# Autodesk Inventor assembly: AxisX
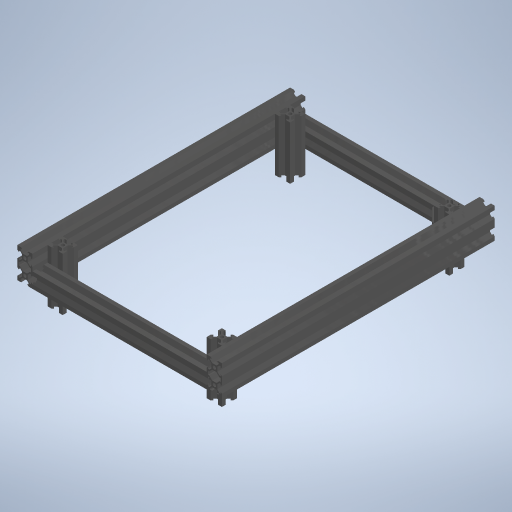
[picture p0: Inventor's stored thumbnail of the model, 512x512]
Saved by Autodesk Inventor 2024.2 (Build 282272000, 272)
## iProperties
Created: 2024-08-26
Part Number: AxisX
Document SubType Name: Assembly
Designer: Admin
Author: Admin
## Documents named in this file (5)
- C:\Users\Admin\Documents\GitHub\ManipuladorCartesiano\DiseñoMecánico\Assemblies\AxisX.iam
- C:\Users\Admin\Documents\GitHub\ManipuladorCartesiano\DiseñoMecánico\Axis\AxisX\AP-X1.ipt
- C:\Users\Admin\Documents\GitHub\ManipuladorCartesiano\DiseñoMecánico\Axis\AxisX\AP-X2.ipt
- C:\Users\Admin\Documents\GitHub\ManipuladorCartesiano\DiseñoMecánico\Axis\AxisX\AP-Support.ipt
- C:\Users\Admin\Documents\GitHub\ManipuladorCartesiano\DiseñoMecánico\AuxiliarPieces\Bracket 2020\CornerBracket2020.ipt
## Components (10 placed, 4 different names)
1. AP-X1:1 — Mate:1, Flush:1, Flush:2, Mate:3, Flush:5, Flush:8, Mate:7, Flush:10, Mate:12
2. AP-X1:2 — Mate:2, Flush:3, Flush:4, Mate:4, Flush:6, Mate:6, Flush:7, Flush:9, Mate:10, Mate:15
3. AP-X2:1 — Mate:3, Mate:4, Flush:5, Flush:6, Mate:5, Mate:8, Mate:13, Flush:11, Flush:12
4. AP-X2:2 — Mate:1, Flush:1, Flush:2, Mate:2, Flush:3, Flush:4, Mate:9, Mate:11
5. AP-Support:1 — Mate:5, Mate:6, Flush:7, Mate:14, Mate:16
6. AP-Support:2 — Flush:9, Mate:9, Mate:10
7. AP-Support:3 — Flush:10, Mate:11, Mate:12
8. AP-Support:4 — Flush:8, Mate:7, Mate:8
9. CornerBracket2020:1 — Mate:15, Mate:16, Flush:12
10. CornerBracket2020:2 — Mate:13, Flush:11, Mate:14
## Relationships (28: Mate 16, Flush 12)
- Mate:1: AP-X1:1 ↔ AP-X2:2
- Flush:1: AP-X1:1 ↔ AP-X2:2
- Flush:2: AP-X1:1 ↔ AP-X2:2
- Mate:2: AP-X1:2 ↔ AP-X2:2
- Flush:3: AP-X1:2 ↔ AP-X2:2
- Flush:4: AP-X1:2 ↔ AP-X2:2
- Mate:3: AP-X1:1 ↔ AP-X2:1
- Mate:4: AP-X1:2 ↔ AP-X2:1
- Flush:5: AP-X1:1 ↔ AP-X2:1
- Flush:6: AP-X1:2 ↔ AP-X2:1
- Mate:5: AP-X2:1 ↔ AP-Support:1
- Mate:6: AP-X1:2 ↔ AP-Support:1
- Flush:7: AP-X1:2 ↔ AP-Support:1
- Flush:8: AP-X1:1 ↔ AP-Support:4
- Mate:7: AP-X1:1 ↔ AP-Support:4
- Mate:8: AP-X2:1 ↔ AP-Support:4
- Flush:9: AP-X1:2 ↔ AP-Support:2
- Mate:9: AP-X2:2 ↔ AP-Support:2
- Mate:10: AP-X1:2 ↔ AP-Support:2
- Flush:10: AP-X1:1 ↔ AP-Support:3
- Mate:11: AP-X2:2 ↔ AP-Support:3
- Mate:12: AP-X1:1 ↔ AP-Support:3
- Mate:13: AP-X2:1 ↔ CornerBracket2020:2
- Flush:11: AP-X2:1 ↔ CornerBracket2020:2
- Mate:14: AP-Support:1 ↔ CornerBracket2020:2
- Mate:15: AP-X1:2 ↔ CornerBracket2020:1
- Mate:16: AP-Support:1 ↔ CornerBracket2020:1
- Flush:12: AP-X2:1 ↔ CornerBracket2020:1
